# Autodesk Inventor assembly: scintillatorPanel
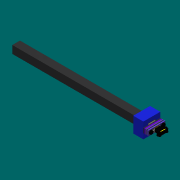
[picture p0: Inventor's stored thumbnail of the model, 180x180]
Saved by Autodesk Inventor 2016 (Build 200138000, 138)
## iProperties
Created: 2016-02-15
Part Number: scintillatorPanel
Document SubType Name: Assembly
Designer: sawai
Author: sawai
## Documents named in this file (6)
- C:\Users\Sawaiz\OneDrive\projects\scintillatorPanel\scintillatorPanel.iam
- C:\Users\Sawaiz\OneDrive\projects\scintillatorPanel\panel.iam
- C:\Users\Sawaiz\OneDrive\projects\scintillatorPanel\mppcSensorInterface\cad\sensorBoard.iam
- C:\Users\Sawaiz\OneDrive\projects\scintillatorPanel\4-40x0.5in.ipt
- C:\Users\Sawaiz\OneDrive\projects\scintillatorPanel\mppcMount.ipt
- C:\Users\Sawaiz\OneDrive\projects\scintillatorPanel\mppcMountClamp.ipt
## Components (6 placed, 5 different names)
1. panel:1 [sub-assembly] — Mate:1, Angle:1, Mate:2, Mate:7, Mate:8, Flush:1, Mate:10
2. sensorBoard:1 [sub-assembly] — Mate:1, Angle:1, Mate:2, Mate:3, Mate:4, Mate:5, Mate:6
3. 4-40x0.5in:1 — Mate:3, Mate:5, Mate:9
4. 4-40x0.5in:2 — Mate:4, Mate:6
5. mppcMount:1 — Mate:7, Mate:8, Flush:1, Mate:9, Flush:2, Flush:3
6. mppcMountClamp:1 — Mate:10, Flush:2, Flush:3
## Relationships (14: Mate 10, Flush 3, Angle 1)
- Mate:1: panel:1 ↔ sensorBoard:1
- Angle:1 (0 deg): panel:1 ↔ sensorBoard:1
- Mate:2: panel:1 ↔ sensorBoard:1
- Mate:3: sensorBoard:1 ↔ 4-40x0.5in:1
- Mate:4: sensorBoard:1 ↔ 4-40x0.5in:2
- Mate:5: sensorBoard:1 ↔ 4-40x0.5in:1
- Mate:6: sensorBoard:1 ↔ 4-40x0.5in:2
- Mate:7: panel:1 ↔ mppcMount:1
- Mate:8: panel:1 ↔ mppcMount:1
- Flush:1: panel:1 ↔ mppcMount:1
- Mate:9: 4-40x0.5in:1 ↔ mppcMount:1
- Mate:10: panel:1 ↔ mppcMountClamp:1
- Flush:2: mppcMount:1 ↔ mppcMountClamp:1
- Flush:3: mppcMount:1 ↔ mppcMountClamp:1
